# Autodesk Inventor assembly: CubeAssembly
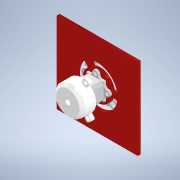
[picture p0: Inventor's stored thumbnail of the model, 180x180]
Saved by Autodesk Inventor 2022 (Build 260153000, 153)
## iProperties
Created: 2022-04-06
Part Number: CubeAssembly
Document SubType Name: Assembly
Designer: awp
Author: awp
## Documents named in this file (8)
- C:\Rice\Junior\Elec327\elec327_rubics_cube\CAD - Copy\CubeAssembly.iam
- C:\Rice\Junior\Elec327\elec327_rubics_cube\CAD - Copy\SpringPotBottom.ipt
- C:\Rice\Junior\Elec327\elec327_rubics_cube\CAD - Copy\Knob.ipt
- C:\Rice\Junior\Elec327\elec327_rubics_cube\CAD - Copy\Pot.ipt
- C:\Rice\Junior\Elec327\elec327_rubics_cube\CAD - Copy\TurnBot.ipt
- C:\Rice\Junior\Elec327\elec327_rubics_cube\CAD - Copy\CubeFace.ipt
- C:\Rice\Junior\Elec327\elec327_rubics_cube\CAD - Copy\CubeKnob.ipt
- C:\Users\awp\Dropbox\BartendingMachine\Flanged Bearing\8mmid12mmod.ipt
## Components (13 placed, 7 different names)
1. SpringPotBottom:1 — Flush:1, Mate:2, Mate:3, Mate:7, Mate:8, Mate:9
2. Knob:1
3. Pot:1 — Flush:1, Mate:2, Mate:3, Mate:4, Mate:5
4. TurnBot:1 — Mate:4, Mate:5
5. CubeFace:1 — Mate:7, Mate:8, Mate:9, Mate:11, Mate:23, Flush:3
6. CubeKnob:1 — Mate:11
7. SpringPotBottom:2 — Mate:24, Mate:25
8. Knob:2 — Mate:26, Mate:28, Mate:29
9. Pot:2
10. TurnBot:2
11. CubeFace:2 — Mate:23, Flush:3, Mate:27
12. CubeKnob:2 — Mate:27, Mate:28, Mate:29
13. 8mmid12mmod:1 — Mate:24, Mate:25, Mate:26
## Relationships (26: Mate 23, Flush 3)
- Flush:1: SpringPotBottom:1 ↔ Pot:1
- Mate:2 (0.1905 mm): SpringPotBottom:1 ↔ Pot:1
- Mate:3 (0.1905 mm): SpringPotBottom:1 ↔ Pot:1
- Mate:4: Pot:1 ↔ TurnBot:1
- Mate:5: Pot:1 ↔ TurnBot:1
- Mate:7: SpringPotBottom:1 ↔ CubeFace:1
- Mate:8: SpringPotBottom:1 ↔ CubeFace:1
- Mate:9: SpringPotBottom:1 ↔ CubeFace:1
- Mate:11: CubeFace:1 ↔ CubeKnob:1
- [Flush]: SpringPotBottom:2 ↔ Pot:2
- [Mate]: SpringPotBottom:2 ↔ Pot:2
- [Mate]: SpringPotBottom:2 ↔ Pot:2
- [Mate]: Pot:2 ↔ TurnBot:2
- [Mate]: Pot:2 ↔ TurnBot:2
- [Mate]: Knob:2 ↔ TurnBot:2
- [Mate]: SpringPotBottom:2 ↔ CubeFace:2
- [Mate]: SpringPotBottom:2 ↔ CubeFace:2
- [Mate]: SpringPotBottom:2 ↔ CubeFace:2
- Mate:23: CubeFace:1 ↔ CubeFace:2
- Flush:3: CubeFace:1 ↔ CubeFace:2
- Mate:24: SpringPotBottom:2 ↔ 8mmid12mmod:1
- Mate:25: SpringPotBottom:2 ↔ 8mmid12mmod:1
- Mate:26: Knob:2 ↔ 8mmid12mmod:1
- Mate:27 (5.08 mm): CubeFace:2 ↔ CubeKnob:2
- Mate:28: Knob:2 ↔ CubeKnob:2
- Mate:29: Knob:2 ↔ CubeKnob:2
## Named parameters: d14_d3 = 0 mm, d15_d4 = 0 mm, d16_d5 = 0 mm, d17_d6 = 0 mm, d18_d7 = 0 mm, d19_d8 = 0 mm, d20_d9 = 0 mm, d24_d1 = 0 mm, d25_d2 = 0 mm
